# Autodesk Inventor assembly: Elevator Lifter
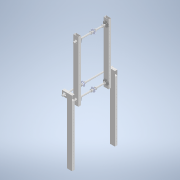
[picture p0: Inventor's stored thumbnail of the model, 180x180]
Saved by Autodesk Inventor 2022 (Build 260153000, 153)
## iProperties
Created: 2021-01-30
Part Number: Elevator Lifter
Document SubType Name: Assembly
Designer: aidan
Author: aidan
## Documents named in this file (10)
- C:\Users\merky\OneDrive\Documents\t3-cad\CAD\2021 Elevator\Elevator Lifter.iam
- C:\Users\merky\OneDrive\Documents\t3-cad\CAD\2021 Elevator\Elevator Versaframe.ipt
- C:\Users\merky\OneDrive\Documents\t3-cad\CAD\2021 Elevator\Elevator VersaframeBacktrack.ipt
- C:\Users\merky\OneDrive\Documents\t3-cad\CAD\2021 Elevator\Generic Elevator Parts\Bearing-Thundershaft.ipt
- C:\Users\merky\OneDrive\Documents\t3-cad\CAD\2021 Elevator\Generic Elevator Parts\Thundershaft-6.ipt
- C:\Users\merky\OneDrive\Documents\t3-cad\CAD\2021 Elevator\Elevator Versaframe2.ipt
- C:\Users\merky\OneDrive\Documents\t3-cad\CAD\2021 Elevator\Generic Elevator Parts\Thundershaft-2.ipt
- C:\Users\merky\OneDrive\Documents\t3-cad\CAD\0.5in Hex Hub.ipt
- C:\Users\merky\OneDrive\Documents\t3-cad\CAD\Generic and Stock\15T Sprocket.ipt
- C:\Users\merky\OneDrive\Documents\t3-cad\CAD\Hex Shaft Collar.ipt
## Components (30 placed, 9 different names)
1. Elevator Versaframe:1 — Mate:23, Flush:34, Flush:35, Mate:26
2. Elevator Versaframe:2 — Mate:24, Flush:36, Flush:37, Mate:28
3. Elevator VersaframeBacktrack:1 — Mate:23, Flush:34, Flush:35, Insert:3, Insert:5
4. Elevator VersaframeBacktrack:2 — Mate:24, Flush:36, Flush:37, Insert:1
5. Bearing-Thundershaft:1 — Insert:1
6. Bearing-Thundershaft:3 — Insert:3
7. Thundershaft-6:1 — Insert:5, Insert:13, Insert:15, Insert:16, Insert:17, Insert:18
8. Elevator Versaframe2:1 — Mate:26, Flush:40, Insert:6, Insert:7, Insert:10
9. Elevator Versaframe2:2 — Mate:28, Flush:40, Insert:8, Insert:9, Insert:11
10. Thundershaft-2:1 — Insert:10, Insert:14, Insert:19, Insert:20, Insert:21, Insert:22
11. Thundershaft-2:2 — Insert:11, Insert:12, Insert:23, Insert:24, Insert:25, Insert:26
12. 0.5in Hex Hub:1 — Insert:6
13. 0.5in Hex Hub:2 — Insert:9
14. 0.5in Hex Hub:3 — Insert:7
15. 0.5in Hex Hub:4 — Insert:8
16. 15T Sprocket:1 — Insert:14
17. 15T Sprocket:2 — Insert:13
18. 15T Sprocket:3 — Insert:12
19. Hex Shaft Collar:1 — Insert:15
20. Hex Shaft Collar:2 — Insert:20
21. Hex Shaft Collar:3 — Insert:23
22. Hex Shaft Collar:4 — Insert:24
23. Hex Shaft Collar:5 — Insert:17
24. Hex Shaft Collar:6 — Insert:19
25. Hex Shaft Collar:7 — Insert:22
26. Hex Shaft Collar:8 — Insert:26
27. Hex Shaft Collar:9 — Insert:16
28. Hex Shaft Collar:10 — Insert:18
29. Hex Shaft Collar:11 — Insert:21
30. Hex Shaft Collar:12 — Insert:25
## Relationships (33: Insert 24, Flush 5, Mate 4)
- Mate:23: Elevator Versaframe:1 ↔ Elevator VersaframeBacktrack:1
- Flush:34: Elevator Versaframe:1 ↔ Elevator VersaframeBacktrack:1
- Flush:35: Elevator Versaframe:1 ↔ Elevator VersaframeBacktrack:1
- Mate:24: Elevator Versaframe:2 ↔ Elevator VersaframeBacktrack:2
- Flush:36: Elevator Versaframe:2 ↔ Elevator VersaframeBacktrack:2
- Flush:37: Elevator Versaframe:2 ↔ Elevator VersaframeBacktrack:2
- Insert:1: Elevator VersaframeBacktrack:2 ↔ Bearing-Thundershaft:1
- Insert:3: Elevator VersaframeBacktrack:1 ↔ Bearing-Thundershaft:3
- Insert:5 (-25.4 mm): Elevator VersaframeBacktrack:1 ↔ Thundershaft-6:1
- Mate:26 (38.1 mm): Elevator Versaframe:1 ↔ Elevator Versaframe2:1
- Mate:28 (38.1 mm): Elevator Versaframe:2 ↔ Elevator Versaframe2:2
- Flush:40: Elevator Versaframe2:1 ↔ Elevator Versaframe2:2
- Insert:6: Elevator Versaframe2:1 ↔ 0.5in Hex Hub:1
- Insert:7: Elevator Versaframe2:1 ↔ 0.5in Hex Hub:3
- Insert:8: Elevator Versaframe2:2 ↔ 0.5in Hex Hub:4
- Insert:9: Elevator Versaframe2:2 ↔ 0.5in Hex Hub:2
- Insert:10 (-20.32 mm): Elevator Versaframe2:1 ↔ Thundershaft-2:1
- Insert:11 (-38.1 mm): Elevator Versaframe2:2 ↔ Thundershaft-2:2
- Insert:12 (-203.2 mm): Thundershaft-2:2 ↔ 15T Sprocket:3
- Insert:13 (-203.2 mm): Thundershaft-6:1 ↔ 15T Sprocket:2
- Insert:14 (203.2 mm): Thundershaft-2:1 ↔ 15T Sprocket:1
- Insert:15 (-63.5 mm): Thundershaft-6:1 ↔ Hex Shaft Collar:1
- Insert:16 (-228.6 mm): Thundershaft-6:1 ↔ Hex Shaft Collar:9
- Insert:17 (-190.5 mm): Thundershaft-6:1 ↔ Hex Shaft Collar:5
- Insert:18 (-63.5 mm): Thundershaft-6:1 ↔ Hex Shaft Collar:10
- Insert:19 (-63.5 mm): Thundershaft-2:1 ↔ Hex Shaft Collar:6
- Insert:20 (-68.58 mm): Thundershaft-2:1 ↔ Hex Shaft Collar:2
- Insert:21 (-177.8 mm): Thundershaft-2:1 ↔ Hex Shaft Collar:11
- Insert:22 (-152.4 mm): Thundershaft-2:1 ↔ Hex Shaft Collar:7
- Insert:23 (-76.2 mm): Thundershaft-2:2 ↔ Hex Shaft Collar:3
- Insert:24 (-76.2 mm): Thundershaft-2:2 ↔ Hex Shaft Collar:4
- Insert:25 (-152.4 mm): Thundershaft-2:2 ↔ Hex Shaft Collar:12
- Insert:26 (-177.8 mm): Thundershaft-2:2 ↔ Hex Shaft Collar:8
